# Autodesk Inventor assembly: arbre_roue
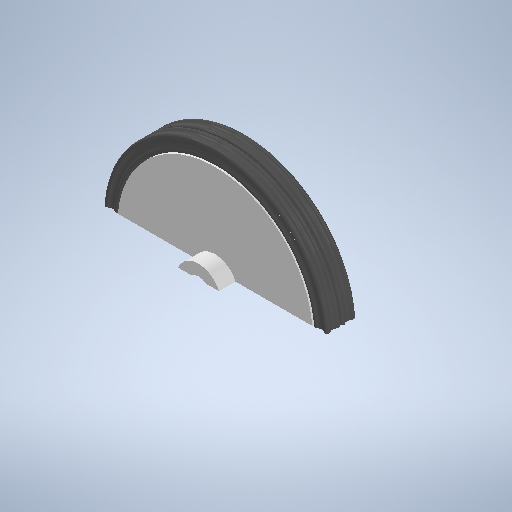
[picture p0: Inventor's stored thumbnail of the model, 512x512]
Saved by Autodesk Inventor 2025.2 (Build 292293000, 293)
## iProperties
Created: 2025-03-27
Part Number: arbre_roue
Document SubType Name: Assembly
Designer: enezl
Author: enezl
## Documents named in this file (4)
- E:\Documents\GitHub\CDFR2025\FIPABOT\inventor\arbre_roue.iam
- E:\Documents\GitHub\CDFR2025\FIPABOT\inventor\arbre_roue.ipt
- E:\Documents\GitHub\CDFR2025\FIPABOT\inventor\roue.ipt
- E:\Documents\GitHub\CDFR2025\FIPABOT\inventor\joint_jf4_libre_202003.ipt
## Components (4 placed, 3 different names)
1. arbre_roue:1 — Logement:1
2. roue:1 — Logement:1, Rotation:1, Rotation:2
3. joint_jf4_libre_202003:1 — Rotation:1
4. joint_jf4_libre_202003:2 — Rotation:2
## Relationships (3: RevoluteJoint 2, Insert 1)
- Logement:1 [Insert]: arbre_roue:1 ↔ roue:1
- Rotation:1 [RevoluteJoint] (-1.1 mm): roue:1 ↔ joint_jf4_libre_202003:1
- Rotation:2 [RevoluteJoint] (-1.1 mm): roue:1 ↔ joint_jf4_libre_202003:2
